# Autodesk Inventor assembly: FullClimbAttatchment
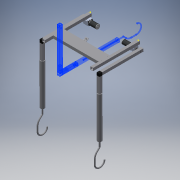
[picture p0: Inventor's stored thumbnail of the model, 180x180]
Saved by Autodesk Inventor 2017 (Build 210142000, 142)
## iProperties
Created: 2020-02-22
Part Number: FullClimbAttatchment
Document SubType Name: Assembly
Designer: S338674153
Author: S338674153
## Documents named in this file (5)
- \\ad.ocdsb.ca\studenthome\3\S338674153\FRC 2020\FullRobotRefactor\Climb\FullClimbAttatchment.iam
- \\ad.ocdsb.ca\studenthome\3\S338674153\FRC 2020\FullRobotRefactor\Climb\Vertical frame Extension 2.ipt
- \\ad.ocdsb.ca\studenthome\3\S338674153\FRC 2020\FullRobotRefactor\Camera\Pi_Camera_Mount_Assembly.iam
- \\ad.ocdsb.ca\studenthome\3\S338674153\FRC 2020\FullRobotRefactor\Motors\VersaPlanetary_v1_Single_Stage_10_1_with_BAG.ipt
- \\ad.ocdsb.ca\studenthome\3\S338674153\FRC 2020\FullRobotRefactor\Climb\ClimbMechanism.iam
## Components (7 placed, 4 different names)
1. Vertical frame Extension 2:1 — Flush:1, Flush:2, Mate:1, Flush:4, Flush:7, Mate:4, Flush:8
2. Vertical frame Extension 2:2 — Flush:1, Flush:2, Mate:1, Mate:2, Flush:3, Flush:5, Mate:3, Flush:6
3. Pi_Camera_Mount_Assembly:1 [sub-assembly] — Mate:2, Flush:3, Flush:4
4. VersaPlanetary_v1_Single_Stage_10_1_with_BAG:1 — Flush:5, Mate:3, Flush:6, Mate:6, Flush:11
5. VersaPlanetary_v1_Single_Stage_10_1_with_BAG:2 — Flush:7, Mate:4, Flush:8, Mate:5, Flush:9
6. ClimbMechanism:1 [sub-assembly] — Mate:6, Flush:10, Flush:11
7. ClimbMechanism:2 [sub-assembly] — Mate:5, Flush:9, Flush:10
## Relationships (17: Flush 11, Mate 6)
- Flush:1: Vertical frame Extension 2:1 ↔ Vertical frame Extension 2:2
- Flush:2: Vertical frame Extension 2:1 ↔ Vertical frame Extension 2:2
- Mate:1 (419.1 mm): Vertical frame Extension 2:1 ↔ Vertical frame Extension 2:2
- Mate:2: Vertical frame Extension 2:2 ↔ Pi_Camera_Mount_Assembly:1
- Flush:3: Vertical frame Extension 2:2 ↔ Pi_Camera_Mount_Assembly:1
- Flush:4 (254 mm): Vertical frame Extension 2:1 ↔ Pi_Camera_Mount_Assembly:1
- Flush:5: Vertical frame Extension 2:2 ↔ VersaPlanetary_v1_Single_Stage_10_1_with_BAG:1
- Mate:3: Vertical frame Extension 2:2 ↔ VersaPlanetary_v1_Single_Stage_10_1_with_BAG:1
- Flush:6 (12.7 mm): Vertical frame Extension 2:2 ↔ VersaPlanetary_v1_Single_Stage_10_1_with_BAG:1
- Flush:7: Vertical frame Extension 2:1 ↔ VersaPlanetary_v1_Single_Stage_10_1_with_BAG:2
- Mate:4: Vertical frame Extension 2:1 ↔ VersaPlanetary_v1_Single_Stage_10_1_with_BAG:2
- Flush:8 (12.7 mm): Vertical frame Extension 2:1 ↔ VersaPlanetary_v1_Single_Stage_10_1_with_BAG:2
- Mate:5: VersaPlanetary_v1_Single_Stage_10_1_with_BAG:2 ↔ ClimbMechanism:2
- Flush:9: VersaPlanetary_v1_Single_Stage_10_1_with_BAG:2 ↔ ClimbMechanism:2
- Mate:6: VersaPlanetary_v1_Single_Stage_10_1_with_BAG:1 ↔ ClimbMechanism:1
- Flush:10: ClimbMechanism:1 ↔ ClimbMechanism:2
- Flush:11: VersaPlanetary_v1_Single_Stage_10_1_with_BAG:1 ↔ ClimbMechanism:1
